# Autodesk Inventor assembly: kiiker_maket
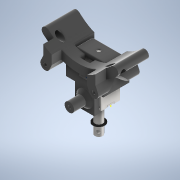
[picture p0: Inventor's stored thumbnail of the model, 180x180]
Saved by Autodesk Inventor 2020 (Build 240168000, 168)
## iProperties
Created: 2024-02-27
Part Number: kiiker_maket
Document SubType Name: Assembly
Designer: 4s
Author: 4s
## Documents named in this file (4)
- C:\Users\4s\Documents\Inventor models\Asterisk\robot_v2\kicker\kiiker_maket.iam
- C:\Users\4s\Documents\Inventor models\Asterisk\robot_v2\kicker\kicker_base_v6_wide.ipt
- C:\Users\4s\Documents\Inventor models\Asterisk\robot_v2\kicker\kicker_head_flat_v4.ipt
- C:\Users\4s\Documents\Inventor models\Solenoid\solenoid.iam
## Components (3 placed, 3 different names)
1. kicker_base_v6_wide:1 — Заподлицо:1, Заподлицо:2, Заподлицо:3, Заподлицо:4, Совмещение:1, Совмещение:2, Совмещение:3, Совмещение:4, Совмещение:6
2. kicker_head_flat_v4:1 — Совмещение:1, Совмещение:2, Совмещение:3, Совмещение:5
3. solenoid:1 [sub-assembly] — Совмещение:4, Совмещение:5, Совмещение:6, Угол:1
## Relationships (11: Mate 6, Flush 4, Angle 1)
- Заподлицо:1 [Flush]: kicker_base_v6_wide:1
- Заподлицо:2 [Flush]: kicker_base_v6_wide:1
- Заподлицо:3 [Flush]: kicker_base_v6_wide:1
- Заподлицо:4 [Flush]: kicker_base_v6_wide:1
- Совмещение:1 [Mate]: kicker_base_v6_wide:1 ↔ kicker_head_flat_v4:1
- Совмещение:2 [Mate]: kicker_base_v6_wide:1 ↔ kicker_head_flat_v4:1
- Совмещение:3 [Mate]: kicker_base_v6_wide:1 ↔ kicker_head_flat_v4:1
- Совмещение:4 [Mate]: kicker_base_v6_wide:1 ↔ solenoid:1
- Совмещение:5 [Mate]: kicker_head_flat_v4:1 ↔ solenoid:1
- Совмещение:6 [Mate]: kicker_base_v6_wide:1 ↔ solenoid:1
- Угол:1 [Angle] (0 deg): solenoid:1
